# Autodesk Inventor assembly: Robot
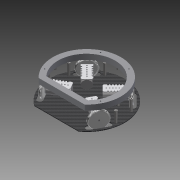
[picture p0: Inventor's stored thumbnail of the model, 180x180]
Saved by Autodesk Inventor 2015 (Build 190159000, 159)
## iProperties
Created: 2016-08-02
Part Number: Robot
Document SubType Name: Assembly
Designer: James Yelland
Author: James Yelland
## Documents named in this file (9)
- C:\Users\James Yelland\git\Layers-2017\Models\Robot.iam
- C:\Users\James Yelland\git\Layers-2017\Models\Bottom Plate.ipt
- C:\Users\James Yelland\git\Layers-2017\Models\Middle Plate.ipt
- C:\Users\James Yelland\git\Layers-2017\Models\Motor Mount Bracket.ipt
- C:\Users\James Yelland\git\Layers-2017\Models\Motor.ipt
- C:\Users\James Yelland\git\Layers-2017\Models\Standoff 35.ipt
- C:\Users\James Yelland\git\Layers-2017\Models\Wheel.ipt
- C:\Users\James Yelland\git\Layers-2017\Models\Standoff 10.ipt
- C:\Users\James Yelland\git\Layers-2017\Models\TSOP Ring.ipt
## Components (24 placed, 8 different names)
1. Bottom Plate:1 — Mate:38, Mate:39, Mate:40
2. Middle Plate:1 — Mate:1, Mate:3, Mate:4, Mate:5, Mate:6, Mate:7, Mate:8, Mate:9, Mate:10, Mate:11, Mate:12, Mate:13, Mate:26, Mate:27, Mate:28, Mate:29, Mate:30, Mate:31, Mate:32, Mate:33, Mate:34, Mate:35, Mate:36, Mate:37, Mate:45, Mate:46, Mate:47, Mate:48, Mate:49, Mate:50
3. Motor Mount Bracket:1 — Mate:5, Mate:10, Mate:11, Mate:15, Mate:24, Mate:25
4. Motor Mount Bracket:2 — Mate:1, Mate:12, Mate:13, Mate:14, Mate:20, Mate:21
5. Motor Mount Bracket:3 — Mate:3, Mate:8, Mate:9, Mate:16, Mate:22, Mate:23
6. Motor Mount Bracket:4 — Mate:4, Mate:6, Mate:7, Mate:17, Mate:18, Mate:19
7. Motor:1 — Mate:15, Mate:24, Mate:25, Mate:44, Flush:4
8. Motor:2 — Mate:17, Mate:18, Mate:19, Mate:43, Flush:3
9. Motor:3 — Mate:16, Mate:22, Mate:23, Flush:1, Mate:41
10. Motor:4 — Mate:14, Mate:20, Mate:21, Mate:42, Flush:2
11. Standoff 35:1 — Mate:31, Mate:32, Mate:40
12. Standoff 35:2 — Mate:30, Mate:33
13. Standoff 35:3 — Mate:29, Mate:34
14. Standoff 35:4 — Mate:28, Mate:35
15. Standoff 35:5 — Mate:27, Mate:36, Mate:38
16. Standoff 35:6 — Mate:26, Mate:37, Mate:39
17. Wheel:1 — Flush:1, Mate:41
18. Wheel:2 — Mate:42, Flush:2
19. Wheel:3 — Mate:43, Flush:3
20. Wheel:4 — Mate:44, Flush:4
21. Standoff 10:1 — Mate:47, Mate:50, Mate:52
22. Standoff 10:2 — Mate:46, Mate:49, Mate:51
23. Standoff 10:3 — Mate:45, Mate:48, Mate:53
24. TSOP Ring:1 — Mate:51, Mate:52, Mate:53
## Relationships (56: Mate 52, Flush 4)
- Mate:1: Middle Plate:1 ↔ Motor Mount Bracket:2
- Mate:3: Middle Plate:1 ↔ Motor Mount Bracket:3
- Mate:4: Middle Plate:1 ↔ Motor Mount Bracket:4
- Mate:5: Middle Plate:1 ↔ Motor Mount Bracket:1
- Mate:6: Middle Plate:1 ↔ Motor Mount Bracket:4
- Mate:7: Middle Plate:1 ↔ Motor Mount Bracket:4
- Mate:8: Middle Plate:1 ↔ Motor Mount Bracket:3
- Mate:9: Middle Plate:1 ↔ Motor Mount Bracket:3
- Mate:10: Middle Plate:1 ↔ Motor Mount Bracket:1
- Mate:11: Middle Plate:1 ↔ Motor Mount Bracket:1
- Mate:12: Middle Plate:1 ↔ Motor Mount Bracket:2
- Mate:13: Middle Plate:1 ↔ Motor Mount Bracket:2
- Mate:14: Motor Mount Bracket:2 ↔ Motor:4
- Mate:15: Motor Mount Bracket:1 ↔ Motor:1
- Mate:16: Motor Mount Bracket:3 ↔ Motor:3
- Mate:17: Motor Mount Bracket:4 ↔ Motor:2
- Mate:18: Motor Mount Bracket:4 ↔ Motor:2
- Mate:19: Motor Mount Bracket:4 ↔ Motor:2
- Mate:20: Motor Mount Bracket:2 ↔ Motor:4
- Mate:21: Motor Mount Bracket:2 ↔ Motor:4
- Mate:22: Motor Mount Bracket:3 ↔ Motor:3
- Mate:23: Motor Mount Bracket:3 ↔ Motor:3
- Mate:24: Motor Mount Bracket:1 ↔ Motor:1
- Mate:25: Motor Mount Bracket:1 ↔ Motor:1
- Mate:26: Middle Plate:1 ↔ Standoff 35:6
- Mate:27: Middle Plate:1 ↔ Standoff 35:5
- Mate:28: Middle Plate:1 ↔ Standoff 35:4
- Mate:29: Middle Plate:1 ↔ Standoff 35:3
- Mate:30: Middle Plate:1 ↔ Standoff 35:2
- Mate:31: Middle Plate:1 ↔ Standoff 35:1
- Mate:32: Middle Plate:1 ↔ Standoff 35:1
- Mate:33: Middle Plate:1 ↔ Standoff 35:2
- Mate:34: Middle Plate:1 ↔ Standoff 35:3
- Mate:35: Middle Plate:1 ↔ Standoff 35:4
- Mate:36: Middle Plate:1 ↔ Standoff 35:5
- Mate:37: Middle Plate:1 ↔ Standoff 35:6
- Mate:38: Bottom Plate:1 ↔ Standoff 35:5
- Mate:39: Bottom Plate:1 ↔ Standoff 35:6
- Mate:40: Bottom Plate:1 ↔ Standoff 35:1
- Flush:1: Motor:3 ↔ Wheel:1
- Mate:41: Motor:3 ↔ Wheel:1
- Mate:42: Motor:4 ↔ Wheel:2
- Flush:2: Motor:4 ↔ Wheel:2
- Mate:43: Motor:2 ↔ Wheel:3
- Flush:3: Motor:2 ↔ Wheel:3
- Mate:44: Motor:1 ↔ Wheel:4
- Flush:4: Motor:1 ↔ Wheel:4
- Mate:45: Middle Plate:1 ↔ Standoff 10:3
- Mate:46: Middle Plate:1 ↔ Standoff 10:2
- Mate:47: Middle Plate:1 ↔ Standoff 10:1
- Mate:48: Middle Plate:1 ↔ Standoff 10:3
- Mate:49: Middle Plate:1 ↔ Standoff 10:2
- Mate:50: Middle Plate:1 ↔ Standoff 10:1
- Mate:51: Standoff 10:2 ↔ TSOP Ring:1
- Mate:52: Standoff 10:1 ↔ TSOP Ring:1
- Mate:53: Standoff 10:3 ↔ TSOP Ring:1
